# Autodesk Inventor assembly: EX_ONE
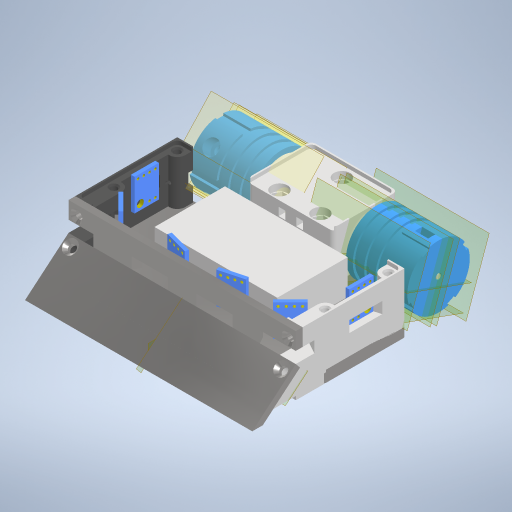
[picture p0: Inventor's stored thumbnail of the model, 512x512]
Saved by Autodesk Inventor 2023 (Build 270158000, 158)
## iProperties
Created: 2025-01-11
Part Number: EX_ONE
Document SubType Name: Assembly
Designer: kamil
Author: kamil
## Documents named in this file (15)
- C:\Users\kamil\Documents\PROJECTS - repos\EX_ONE_minisumo\mechanics\inventor_parts\EX_ONE.iam
- C:\Users\kamil\Documents\PROJECTS - repos\EX_ONE_minisumo\mechanics\inventor_parts\faulhaber_motor.ipt
- C:\Users\kamil\Documents\PROJECTS - repos\EX_ONE_minisumo\mechanics\inventor_parts\motors_mount.ipt
- C:\Users\kamil\Documents\PROJECTS - repos\EX_ONE_minisumo\mechanics\inventor_parts\kolo_tetsowe.ipt
- C:\Users\kamil\Documents\PROJECTS - repos\EX_ONE_minisumo\mechanics\inventor_parts\podstawa.ipt
- C:\Users\kamil\Documents\PROJECTS - repos\EX_ONE_minisumo\mechanics\inventor_parts\nóź.ipt
- C:\Users\kamil\Documents\PROJECTS - repos\EX_ONE_minisumo\mechanics\inventor_parts\TOF_VL53L0X (1).ipt
- C:\Users\kamil\Documents\PROJECTS - repos\EX_ONE_minisumo\mechanics\inventor_parts\ściana.ipt
- C:\Users\kamil\Documents\PROJECTS - repos\EX_ONE_minisumo\mechanics\inventor_parts\przod.ipt
- C:\Users\kamil\Documents\PROJECTS - repos\EX_ONE_minisumo\mechanics\inventor_parts\oslona.ipt
- C:\Users\kamil\Documents\PROJECTS - repos\EX_ONE_minisumo\mechanics\inventor_parts\pokrywa.ipt
- C:\Users\kamil\Documents\PROJECTS - repos\EX_ONE_minisumo\mechanics\inventor_parts\belka.ipt
- C:\Users\kamil\Documents\PROJECTS - repos\EX_ONE_minisumo\mechanics\inventor_parts\pcb_czujnik.ipt
- C:\Users\kamil\Documents\PROJECTS - repos\EX_ONE_minisumo\mechanics\inventor_parts\li_po_400mAh.ipt
- C:\Users\kamil\Documents\PROJECTS - repos\EX_ONE_minisumo\mechanics\inventor_parts\sciana_left.ipt
## Components (21 placed, 14 different names)
1. faulhaber_motor:1 — Zestawiające:31
2. faulhaber_motor:2 — Zestawiające:30
3. motors_mount:1 — Zestawiające:29, Zestawiające:30, Zestawiające:31, Równoległe:53
4. kolo_tetsowe:1
5. nóź:1 — Zestawiające:48
6. kolo_tetsowe:2
7. ściana:1 — Zestawiające:18, Równoległe:21, Zestawiające:19, Równoległe:22, Zestawiające:28, Równoległe:27, Równoległe:28, Równoległe:30, Zestawiające:34, Kątowe:9, Równoległe:35, Zestawiające:35
8. przod:1 — Zestawiające:18, Równoległe:21, Zestawiające:19
9. oslona:1 — Równoległe:22, Zestawiające:41
10. pokrywa:1
11. belka:1 — Zestawiające:28, Równoległe:27, Równoległe:28
12. podstawa:1 — Zestawiające:29, Równoległe:30, Zestawiające:40, Zestawiające:47, Równoległe:54
13. pcb_czujnik:1 — Zestawiające:34, Kątowe:9, Równoległe:35, Zestawiające:35
14. li_po_400mAh:1 — Zestawiające:40, Zestawiające:41, Równoległe:53
15. TOF_VL53L0X (1):8
16. TOF_VL53L0X (1):9 — Równoległe:52
17. TOF_VL53L0X (1):10
18. TOF_VL53L0X (1):11 — Równoległe:52
19. TOF_VL53L0X (1):12
20. TOF_VL53L0X (1):13
21. sciana_left:1 — Zestawiające:47, Zestawiające:48, Równoległe:54
## Relationships (22: Mate 12, Flush 9, Angle 1)
- Zestawiające:18 [Mate]: ściana:1 ↔ przod:1
- Równoległe:21 [Flush]: ściana:1 ↔ przod:1
- Zestawiające:19 [Mate]: ściana:1 ↔ przod:1
- Równoległe:22 [Flush]: ściana:1 ↔ oslona:1
- Zestawiające:28 [Mate]: ściana:1 ↔ belka:1
- Równoległe:27 [Flush]: ściana:1 ↔ belka:1
- Równoległe:28 [Flush]: ściana:1 ↔ belka:1
- Zestawiające:29 [Mate]: motors_mount:1 ↔ podstawa:1
- Równoległe:30 [Flush]: ściana:1 ↔ podstawa:1
- Zestawiające:30 [Mate]: faulhaber_motor:2 ↔ motors_mount:1
- Zestawiające:31 [Mate]: faulhaber_motor:1 ↔ motors_mount:1
- Zestawiające:34 [Mate]: ściana:1 ↔ pcb_czujnik:1
- Kątowe:9 [Angle] (0 deg): ściana:1 ↔ pcb_czujnik:1
- Równoległe:35 [Flush]: ściana:1 ↔ pcb_czujnik:1
- Zestawiające:35 [Mate] (0.5 mm): ściana:1 ↔ pcb_czujnik:1
- Zestawiające:40 [Mate]: podstawa:1 ↔ li_po_400mAh:1
- Zestawiające:41 [Mate]: oslona:1 ↔ li_po_400mAh:1
- Równoległe:52 [Flush]: TOF_VL53L0X (1):9 ↔ TOF_VL53L0X (1):11
- Równoległe:53 [Flush] (8 mm): motors_mount:1 ↔ li_po_400mAh:1
- Zestawiające:47 [Mate]: podstawa:1 ↔ sciana_left:1
- Zestawiające:48 [Mate]: nóź:1 ↔ sciana_left:1
- Równoległe:54 [Flush]: podstawa:1 ↔ sciana_left:1
